# Autodesk Inventor assembly: arm TOPLEVEL
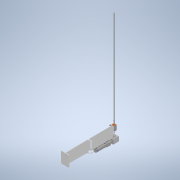
[picture p0: Inventor's stored thumbnail of the model, 180x180]
Saved by Autodesk Inventor 2021 (Build 250183000, 183)
## iProperties
Created: 2021-03-29
Part Number: arm TOPLEVEL
Document SubType Name: Assembly
Designer: Work
Author: Work
## Documents named in this file (17)
- C:\Users\Work\OneDrive - Brookhaven National Laboratory\Daniels, William intern HPR station\Arm\arm TOPLEVEL.iam
- C:\Users\Work\OneDrive - Brookhaven National Laboratory\Daniels, William intern HPR station\Arm\arm shaft SUB.iam
- C:\Users\Work\OneDrive - Brookhaven National Laboratory\Daniels, William intern HPR station\Arm\arm mount.ipt
- C:\Users\Work\OneDrive - Brookhaven National Laboratory\Daniels, William intern HPR station\Arm\arm stage 1.ipt
- C:\Users\Work\OneDrive - Brookhaven National Laboratory\Daniels, William intern HPR station\Arm\stage2.ipt
- C:\Users\Work\OneDrive - Brookhaven National Laboratory\Daniels, William intern HPR station\Arm\arm attachments SUB.iam
- C:\Users\Work\OneDrive - Brookhaven National Laboratory\Daniels, William intern HPR station\Arm\lock ring 2 supp.ipt
- C:\Users\Work\OneDrive - Brookhaven National Laboratory\Daniels, William intern HPR station\Arm\lock ring 2.ipt
- C:\Users\Work\OneDrive - Brookhaven National Laboratory\Daniels, William intern HPR station\Arm\lock ring 1 supp.ipt
- C:\Users\Work\OneDrive - Brookhaven National Laboratory\Daniels, William intern HPR station\Arm\lock ring 1.ipt
- C:\Users\Work\OneDrive - Brookhaven National Laboratory\Daniels, William intern HPR station\dimensions.xlsx
- C:\Users\Work\OneDrive - Brookhaven National Laboratory\Daniels, William intern HPR station\Arm\arm TOPLEVEL\AIP\FEA\dk6k82h34.fins
- C:\Users\Work\OneDrive - Brookhaven National Laboratory\Daniels, William intern HPR station\Arm\arm TOPLEVEL\AIP\FEA\dk6k82h34.fsat
- C:\Users\Work\OneDrive - Brookhaven National Laboratory\Daniels, William intern HPR station\Arm\arm TOPLEVEL\AIP\FEA\dk6k82h34.ftes
- C:\Users\Work\OneDrive - Brookhaven National Laboratory\Daniels, William intern HPR station\Arm\arm TOPLEVEL\AIP\FEA\dk6k82h34.fwiz
- C:\Users\Work\OneDrive - Brookhaven National Laboratory\Daniels, William intern HPR station\Arm\arm TOPLEVEL\AIP\FEA\dk6k82hhc.fmsh
- C:\Users\Work\OneDrive - Brookhaven National Laboratory\Daniels, William intern HPR station\Arm\arm TOPLEVEL\AIP\FEA\dk6k82hhd.fres
## Components (10 placed, 9 different names)
1. arm shaft SUB:1 [sub-assembly] — Rotational:1, Rigid:1
2. arm mount:1 — Rotational:1, Rigid:7
3. arm stage 1:1 — Rigid:1, Rotational:3, Rigid:6
4. arm shaft SUB:2 [sub-assembly] — Rotational:3, Rigid:3
5. stage2:1 — Rigid:3, Rigid:4
6. arm attachments SUB:1 [sub-assembly] — Rigid:4
7. lock ring 2 supp:1 — Rigid:5, Rigid:6
8. lock ring 2:1 — Rigid:5
9. lock ring 1 supp:2 — Rigid:7, Rigid:8
10. lock ring 1:1 — Rigid:8
## Relationships (9: WeldJoint 7, RevoluteJoint 2)
- Rotational:1 [RevoluteJoint]: arm shaft SUB:1 ↔ arm mount:1
- Rigid:1 [WeldJoint]: arm shaft SUB:1 ↔ arm stage 1:1
- Rotational:3 [RevoluteJoint]: arm stage 1:1 ↔ arm shaft SUB:2
- Rigid:3 [WeldJoint]: arm shaft SUB:2 ↔ stage2:1
- Rigid:4 [WeldJoint]: stage2:1 ↔ arm attachments SUB:1
- Rigid:5 [WeldJoint]: lock ring 2 supp:1 ↔ lock ring 2:1
- Rigid:6 [WeldJoint]: arm stage 1:1 ↔ lock ring 2 supp:1
- Rigid:7 [WeldJoint]: arm mount:1 ↔ lock ring 1 supp:2
- Rigid:8 [WeldJoint]: lock ring 1 supp:2 ↔ lock ring 1:1
## Named parameters: height = 203.2 mm, shaftDiam = 6.35 mm, shaftSpace = 1.5875 mm, stageSpace = 2.54 mm, stageAngle = 15 deg, sa_0 = 980.999, groundActu = 304.8 mm, capThickness = 3.175 mm, baseDepth = 254 mm, baseWidth = 1066.8 mm, actuHieght = 1800 mm, stockHeight = 50.8 mm, stockWidth = 76.2 mm, stockGuage = 3.175 mm, stockRad = 9.525 mm, sup1Ang = 22.619865 deg, sup1Len = 660.4 mm, supVertLen = 955.13561 mm, sup2Ang = 8.959949 deg, sup2Len = 2079.37366 mm, supSideAng = 19.376933 deg, supSideLen = 1531.12879 mm, FlangeDiam = 12.7 mm, bearingDiam = 9.5504 mm, FlangeDepth = 1.5875 mm, smallFilet = 0.39687 mm, thickness = 12.7 mm, ringDiam = 96.46608 mm
note: some values were not read from the file. Shown as the stored number, unit unknown: "sa_0".
